# Autodesk Inventor assembly: Drivebase AM14U4 Square 28inx28in v411
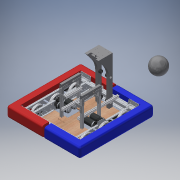
[picture p0: Inventor's stored thumbnail of the model, 180x180]
Saved by Autodesk Inventor 2018 (Build 220112000, 112)
## iProperties
Created: 2020-01-28
Part Number: Drivebase AM14U4 Square 28inx28in v411
Document SubType Name: Assembly
Designer: Weeb No1
Sending System: Autodesk Translation Framework v8.12.0.6
Preprocessor: ST-DEVELOPER v18
Title: /Users/GabG/Documents/GitHub/2020CAD/New Gabriel Shooter/Drivebase AM14U4 Square 28inx28in v41.step
## Documents named in this file (18)
- C:\Users\Weeb No1\Documents\GitHub\2020CAD\Gabriel Inventor Files (Shooter, Drivebase)\Drivebase Assembly\Main Assembly\Drivebase AM14U4 Square 28inx28in v411.iam
- C:\Users\Weeb No1\Documents\GitHub\2020CAD\Gabriel Inventor Files (Shooter, Drivebase)\Drivebase Assembly\Part Files\AM14U4 Square Half.iam
- C:\Users\Weeb No1\Documents\GitHub\2020CAD\Gabriel Inventor Files (Shooter, Drivebase)\Drivebase Assembly\Part Files\AM14U4 Square Half_1.iam
- C:\Users\Weeb No1\Documents\GitHub\2020CAD\Gabriel Inventor Files (Shooter, Drivebase)\Drivebase Assembly\Part Files\Placeholder Belly Pan.ipt
- C:\Users\Weeb No1\Documents\GitHub\2020CAD\Gabriel Inventor Files (Shooter, Drivebase)\Drivebase Assembly\Part Files\10-24 Washer.ipt
- C:\Users\Weeb No1\Documents\GitHub\2020CAD\Gabriel Inventor Files (Shooter, Drivebase)\Drivebase Assembly\Part Files\Bumper Assembly.iam
- C:\Users\Weeb No1\Documents\GitHub\2020CAD\Gabriel Inventor Files (Shooter, Drivebase)\Drivebase Assembly\Part Files\Bumper Assembly_1.iam
- C:\Users\Weeb No1\Documents\GitHub\2020CAD\Gabriel Inventor Files (Shooter, Drivebase)\Drivebase Assembly\Part Files\95335A503_METRIC QUICK-RELEASE PIN.ipt
- C:\Users\Weeb No1\Documents\GitHub\2020CAD\Gabriel Inventor Files (Shooter, Drivebase)\Drivebase Assembly\Part Files\8020 1010 x 19 v2.ipt
- C:\Users\Weeb No1\Documents\GitHub\2020CAD\Gabriel Inventor Files (Shooter, Drivebase)\Drivebase Assembly\Part Files\8020 1010 x 11 5 v2.ipt
- C:\Users\Weeb No1\Documents\GitHub\2020CAD\Gabriel Inventor Files (Shooter, Drivebase)\Drivebase Assembly\Part Files\1x2 9in 1_16_ Beam v7.ipt
- C:\Users\Weeb No1\Documents\GitHub\2020CAD\Gabriel Inventor Files (Shooter, Drivebase)\Drivebase Assembly\Part Files\L-Guesset v1.ipt
- C:\Users\Weeb No1\Documents\GitHub\2020CAD\Gabriel Inventor Files (Shooter, Drivebase)\Drivebase Assembly\Part Files\L-Bracket v1.ipt
- C:\Users\Weeb No1\Documents\GitHub\2020CAD\Gabriel Inventor Files (Shooter, Drivebase)\Drivebase Assembly\Part Files\Component52.ipt
- C:\Users\Weeb No1\Documents\GitHub\2020CAD\Gabriel Inventor Files (Shooter, Drivebase)\Drivebase Assembly\Part Files\8020 1010 x 8 7_8 v6.ipt
- C:\Users\Weeb No1\Documents\GitHub\2020CAD\Gabriel Inventor Files (Shooter, Drivebase)\Drivebase Assembly\Part Files\am-2986 FR8ZZ Hex Bearing v1.ipt
- C:\Users\Weeb No1\Documents\GitHub\2020CAD\Gabriel Inventor Files (Shooter, Drivebase)\Drivebase Assembly\Part Files\Clamping_Shaft_Collar_-_1_2_Hex_ID_217-2737 v1.ipt
- C:\Users\Weeb No1\Documents\GitHub\2020CAD\Gabriel Inventor Files (Shooter, Drivebase)\3D Printed Curve Assembly\Main Assembly\Solid Curve 3D Print v25.iam
## Components (54 placed, 17 different names)
1. AM14U4 Square Half:1 [sub-assembly] — Mate:1, Flush:2, Flush:1, Mate:2, Flush:4, Flush:3, Mate:62, Mate:63, Flush:42, Mate:64, Mate:65, Flush:43, Mate:69, Mate:70, Mate:71, Mate:75, Mate:76, Mate:77, Mate:82, Mate:83, Mate:84, Mate:85, Mate:91, Mate:92, Mate:96, Mate:97
2. AM14U4 Square Half_1:1 [sub-assembly] — Mate:66, Mate:67, Mate:68, Mate:72, Mate:73, Mate:74, Mate:78, Mate:79, Mate:80, Mate:81, Mate:93, Mate:94, Mate:95, Mate:98
3. Placeholder Belly Pan:1 — Mate:21, Mate:59, Mate:22, Mate:58, Mate:86, Mate:91, Mate:92, Mate:93, Mate:94, Mate:95, Mate:96, Mate:97, Mate:98, Mate:99, Mate:100, Mate:101, Mate:102, Mate:103, Mate:104, Mate:105, Mate:106
4. 10-24 Washer:1 — Mate:101
5. 10-24 Washer:2 — Mate:102
6. 10-24 Washer:3 — Mate:100
7. 10-24 Washer:4 — Mate:99
8. 10-24 Washer:5 — Mate:106
9. 10-24 Washer:6 — Mate:105
10. 10-24 Washer:7 — Mate:104
11. 10-24 Washer:8 — Mate:103
12. Bumper Assembly:1 [sub-assembly] — Mate:72, Mate:73, Mate:74, Mate:75, Mate:76, Mate:77
13. Bumper Assembly_1:1 [sub-assembly] — Mate:66, Mate:67, Mate:68, Mate:69, Mate:70, Mate:71
14. 95335A503_METRIC QUICK-RELEASE PIN:1 — Mate:82
15. 95335A503_METRIC QUICK-RELEASE PIN:2 — Mate:83
16. 95335A503_METRIC QUICK-RELEASE PIN:3 — Mate:85
17. 95335A503_METRIC QUICK-RELEASE PIN:4 — Mate:84
18. 95335A503_METRIC QUICK-RELEASE PIN:5 — Mate:78
19. 95335A503_METRIC QUICK-RELEASE PIN:6 — Mate:79
20. 95335A503_METRIC QUICK-RELEASE PIN:7 — Mate:80
21. 95335A503_METRIC QUICK-RELEASE PIN:8 — Mate:81
22. 8020 1010 x 19 v2:1 — Mate:1, Flush:2, Flush:1, Flush:17, Mate:20, Mate:19, Mate:87, Mate:110
23. 8020 1010 x 19 v2:2 — Mate:2, Flush:4, Flush:3, Mate:60, Flush:41, Mate:61, Mate:88, Mate:108
24. 8020 1010 x 11 5 v2:1 — Mate:21, Flush:17, Mate:20, Mate:18, Flush:16, Flush:15, Flush:18, Mate:25, Mate:109, Flush:45
25. 8020 1010 x 11 5 v2:2 — Mate:60, Flush:41, Mate:59, Flush:39, Flush:38, Mate:56, Mate:55, Flush:23, Mate:32, Mate:107, Flush:44
26. 8020 1010 x 11 5 v2:3 — Mate:22, Mate:19, Flush:14, Flush:13, Mate:17, Flush:21, Mate:29
27. 1x2 9in 1_16_ Beam v7:1 — Mate:18, Flush:16, Flush:15, Flush:14, Flush:13, Mate:17, Mate:8, Mate:7, Mate:6, Flush:8, Flush:7, Mate:14, Mate:13, Mate:12, Flush:12, Flush:11, Flush:32, Flush:31, Mate:5, Mate:4, Mate:3, Flush:6, Flush:5, Mate:11, Mate:10, Mate:9, Flush:10, Flush:9, Mate:16, Mate:15
28. 8020 1010 x 11 5 v2:4 — Mate:61, Mate:58, Flush:40, Flush:37, Mate:57, Flush:28, Mate:37
29. 1x2 9in 1_16_ Beam v7:2 — Flush:40, Flush:39, Flush:38, Flush:37, Mate:57, Mate:56, Mate:55, Flush:34, Flush:33, Mate:51, Mate:50, Mate:49, Flush:36, Flush:35, Mate:54, Mate:53, Mate:52, Mate:48, Mate:47, Mate:46, Flush:30, Flush:29, Mate:45, Mate:44, Mate:43, Mate:40, Mate:39
30. L-Guesset v1:1 — Flush:18, Mate:25, Flush:19, Mate:27, Mate:26, Mate:24, Mate:23
31. L-Bracket v1:1 — Flush:19, Mate:27, Mate:26, Flush:20, Mate:28
32. L-Guesset v1:2 — Flush:23, Mate:32, Flush:26, Mate:34, Flush:24, Mate:33
33. L-Bracket v1:2 — Flush:26, Mate:34, Flush:25, Mate:35
34. L-Guesset v1:3 — Mate:8, Mate:7, Mate:6, Flush:8, Flush:7
35. L-Guesset v1:4 — Mate:14, Mate:13, Mate:12, Flush:12, Flush:11
36. L-Guesset v1:5 — Flush:34, Flush:33, Mate:51, Mate:50, Mate:49
37. L-Guesset v1:6 — Flush:36, Flush:35, Mate:54, Mate:53, Mate:52
38. L-Guesset v1:7 — Flush:32, Flush:31, Mate:5, Mate:4, Mate:3, Flush:6, Flush:5
39. L-Guesset v1:8 — Mate:11, Mate:10, Mate:9, Flush:10, Flush:9
40. L-Guesset v1:9 — Mate:48, Mate:47, Mate:46
41. L-Guesset v1:10 — Flush:30, Flush:29, Mate:45, Mate:44, Mate:43
42. L-Bracket v1:3 — Mate:107, Mate:108, Flush:44
43. L-Bracket v1:4 — Mate:109, Mate:110, Flush:45
44. Component52:1
45. L-Guesset v1:11 — Flush:21, Mate:29, Flush:22, Mate:31, Mate:30
46. L-Guesset v1:12 — Flush:28, Mate:37, Flush:27, Mate:38, Mate:36
47. L-Bracket v1:7 — Mate:62, Mate:63, Flush:42, Mate:89
48. L-Bracket v1:8 — Mate:64, Mate:65, Flush:43, Mate:90
49. 8020 1010 x 8 7_8 v6:1 — Flush:27, Mate:38, Mate:36, Flush:25, Mate:35, Flush:24, Mate:33
50. 8020 1010 x 8 7_8 v6:2 — Flush:22, Mate:31, Mate:30, Flush:20, Mate:28, Mate:24, Mate:23
51. am-2986 FR8ZZ Hex Bearing v1:1 — Mate:40, Mate:39, Mate:42, Mate:41
52. Clamping_Shaft_Collar_-_1_2_Hex_ID_217-2737 v1:1 — Mate:42, Mate:41
53. am-2986 FR8ZZ Hex Bearing v1:2 — Mate:16, Mate:15
54. Solid Curve 3D Print v25:1 [sub-assembly] — Mate:86, Mate:87, Mate:88, Mate:89, Mate:90
## Relationships (155: Mate 110, Flush 45)
- Mate:1: AM14U4 Square Half:1 ↔ 8020 1010 x 19 v2:1
- Flush:2 (247.65 mm): AM14U4 Square Half:1 ↔ 8020 1010 x 19 v2:1
- Flush:1: AM14U4 Square Half:1 ↔ 8020 1010 x 19 v2:1
- Mate:2: AM14U4 Square Half:1 ↔ 8020 1010 x 19 v2:2
- Flush:4 (247.65 mm): AM14U4 Square Half:1 ↔ 8020 1010 x 19 v2:2
- Flush:3: AM14U4 Square Half:1 ↔ 8020 1010 x 19 v2:2
- Mate:21: Placeholder Belly Pan:1 ↔ 8020 1010 x 11 5 v2:1
- Flush:17 (9.525 mm): 8020 1010 x 19 v2:1 ↔ 8020 1010 x 11 5 v2:1
- Mate:20: 8020 1010 x 19 v2:1 ↔ 8020 1010 x 11 5 v2:1
- Mate:60: 8020 1010 x 19 v2:2 ↔ 8020 1010 x 11 5 v2:2
- Flush:41 (9.525 mm): 8020 1010 x 19 v2:2 ↔ 8020 1010 x 11 5 v2:2
- Mate:59: Placeholder Belly Pan:1 ↔ 8020 1010 x 11 5 v2:2
- Mate:22: Placeholder Belly Pan:1 ↔ 8020 1010 x 11 5 v2:3
- Mate:19: 8020 1010 x 19 v2:1 ↔ 8020 1010 x 11 5 v2:3
- Mate:18: 8020 1010 x 11 5 v2:1 ↔ 1x2 9in 1_16_ Beam v7:1
- Flush:16: 8020 1010 x 11 5 v2:1 ↔ 1x2 9in 1_16_ Beam v7:1
- Flush:15: 8020 1010 x 11 5 v2:1 ↔ 1x2 9in 1_16_ Beam v7:1
- Flush:14: 8020 1010 x 11 5 v2:3 ↔ 1x2 9in 1_16_ Beam v7:1
- Flush:13: 8020 1010 x 11 5 v2:3 ↔ 1x2 9in 1_16_ Beam v7:1
- Mate:17: 8020 1010 x 11 5 v2:3 ↔ 1x2 9in 1_16_ Beam v7:1
- Mate:61: 8020 1010 x 19 v2:2 ↔ 8020 1010 x 11 5 v2:4
- Mate:58: Placeholder Belly Pan:1 ↔ 8020 1010 x 11 5 v2:4
- Flush:40: 8020 1010 x 11 5 v2:4 ↔ 1x2 9in 1_16_ Beam v7:2
- Flush:39: 8020 1010 x 11 5 v2:2 ↔ 1x2 9in 1_16_ Beam v7:2
- Flush:38: 8020 1010 x 11 5 v2:2 ↔ 1x2 9in 1_16_ Beam v7:2
- Flush:37: 8020 1010 x 11 5 v2:4 ↔ 1x2 9in 1_16_ Beam v7:2
- Mate:57: 8020 1010 x 11 5 v2:4 ↔ 1x2 9in 1_16_ Beam v7:2
- Mate:56: 8020 1010 x 11 5 v2:2 ↔ 1x2 9in 1_16_ Beam v7:2
- Mate:55: 8020 1010 x 11 5 v2:2 ↔ 1x2 9in 1_16_ Beam v7:2
- Flush:18: 8020 1010 x 11 5 v2:1 ↔ L-Guesset v1:1
- Mate:25: 8020 1010 x 11 5 v2:1 ↔ L-Guesset v1:1
- Flush:19: L-Guesset v1:1 ↔ L-Bracket v1:1
- Mate:27: L-Guesset v1:1 ↔ L-Bracket v1:1
- Mate:26: L-Guesset v1:1 ↔ L-Bracket v1:1
- Flush:23: 8020 1010 x 11 5 v2:2 ↔ L-Guesset v1:2
- Mate:32: 8020 1010 x 11 5 v2:2 ↔ L-Guesset v1:2
- Flush:26: L-Guesset v1:2 ↔ L-Bracket v1:2
- Mate:34: L-Guesset v1:2 ↔ L-Bracket v1:2
- Mate:8: 1x2 9in 1_16_ Beam v7:1 ↔ L-Guesset v1:3
- Mate:7: 1x2 9in 1_16_ Beam v7:1 ↔ L-Guesset v1:3
- Mate:6: 1x2 9in 1_16_ Beam v7:1 ↔ L-Guesset v1:3
- Flush:8: 1x2 9in 1_16_ Beam v7:1 ↔ L-Guesset v1:3
- Flush:7: 1x2 9in 1_16_ Beam v7:1 ↔ L-Guesset v1:3
- Mate:14: 1x2 9in 1_16_ Beam v7:1 ↔ L-Guesset v1:4
- Mate:13: 1x2 9in 1_16_ Beam v7:1 ↔ L-Guesset v1:4
- Mate:12: 1x2 9in 1_16_ Beam v7:1 ↔ L-Guesset v1:4
- Flush:12: 1x2 9in 1_16_ Beam v7:1 ↔ L-Guesset v1:4
- Flush:11: 1x2 9in 1_16_ Beam v7:1 ↔ L-Guesset v1:4
- Flush:34: 1x2 9in 1_16_ Beam v7:2 ↔ L-Guesset v1:5
- Flush:33: 1x2 9in 1_16_ Beam v7:2 ↔ L-Guesset v1:5
- Mate:51: 1x2 9in 1_16_ Beam v7:2 ↔ L-Guesset v1:5
- Mate:50: 1x2 9in 1_16_ Beam v7:2 ↔ L-Guesset v1:5
- Mate:49: 1x2 9in 1_16_ Beam v7:2 ↔ L-Guesset v1:5
- Flush:36: 1x2 9in 1_16_ Beam v7:2 ↔ L-Guesset v1:6
- Flush:35: 1x2 9in 1_16_ Beam v7:2 ↔ L-Guesset v1:6
- Mate:54: 1x2 9in 1_16_ Beam v7:2 ↔ L-Guesset v1:6
- Mate:53: 1x2 9in 1_16_ Beam v7:2 ↔ L-Guesset v1:6
- Mate:52: 1x2 9in 1_16_ Beam v7:2 ↔ L-Guesset v1:6
- Flush:32: 1x2 9in 1_16_ Beam v7:1 ↔ L-Guesset v1:7
- Flush:31: 1x2 9in 1_16_ Beam v7:1 ↔ L-Guesset v1:7
- Mate:5: 1x2 9in 1_16_ Beam v7:1 ↔ L-Guesset v1:7
- Mate:4: 1x2 9in 1_16_ Beam v7:1 ↔ L-Guesset v1:7
- Mate:3: 1x2 9in 1_16_ Beam v7:1 ↔ L-Guesset v1:7
- Flush:6: 1x2 9in 1_16_ Beam v7:1 ↔ L-Guesset v1:7
- Flush:5: 1x2 9in 1_16_ Beam v7:1 ↔ L-Guesset v1:7
- Mate:11: 1x2 9in 1_16_ Beam v7:1 ↔ L-Guesset v1:8
- Mate:10: 1x2 9in 1_16_ Beam v7:1 ↔ L-Guesset v1:8
- Mate:9: 1x2 9in 1_16_ Beam v7:1 ↔ L-Guesset v1:8
- Flush:10: 1x2 9in 1_16_ Beam v7:1 ↔ L-Guesset v1:8
- Flush:9: 1x2 9in 1_16_ Beam v7:1 ↔ L-Guesset v1:8
- Mate:48: 1x2 9in 1_16_ Beam v7:2 ↔ L-Guesset v1:9
- Mate:47: 1x2 9in 1_16_ Beam v7:2 ↔ L-Guesset v1:9
- Mate:46: 1x2 9in 1_16_ Beam v7:2 ↔ L-Guesset v1:9
- Flush:30: 1x2 9in 1_16_ Beam v7:2 ↔ L-Guesset v1:10
- Flush:29: 1x2 9in 1_16_ Beam v7:2 ↔ L-Guesset v1:10
- Mate:45: 1x2 9in 1_16_ Beam v7:2 ↔ L-Guesset v1:10
- Mate:44: 1x2 9in 1_16_ Beam v7:2 ↔ L-Guesset v1:10
- Mate:43: 1x2 9in 1_16_ Beam v7:2 ↔ L-Guesset v1:10
- Flush:21: 8020 1010 x 11 5 v2:3 ↔ L-Guesset v1:11
- Mate:29: 8020 1010 x 11 5 v2:3 ↔ L-Guesset v1:11
- Flush:28: 8020 1010 x 11 5 v2:4 ↔ L-Guesset v1:12
- Mate:37: 8020 1010 x 11 5 v2:4 ↔ L-Guesset v1:12
- Flush:27: L-Guesset v1:12 ↔ 8020 1010 x 8 7_8 v6:1
- Mate:38: L-Guesset v1:12 ↔ 8020 1010 x 8 7_8 v6:1
- Mate:36: L-Guesset v1:12 ↔ 8020 1010 x 8 7_8 v6:1
- Flush:25: L-Bracket v1:2 ↔ 8020 1010 x 8 7_8 v6:1
- Mate:35: L-Bracket v1:2 ↔ 8020 1010 x 8 7_8 v6:1
- Flush:24: L-Guesset v1:2 ↔ 8020 1010 x 8 7_8 v6:1
- Mate:33: L-Guesset v1:2 ↔ 8020 1010 x 8 7_8 v6:1
- Flush:22: L-Guesset v1:11 ↔ 8020 1010 x 8 7_8 v6:2
- Mate:31: L-Guesset v1:11 ↔ 8020 1010 x 8 7_8 v6:2
- Mate:30: L-Guesset v1:11 ↔ 8020 1010 x 8 7_8 v6:2
- Flush:20: L-Bracket v1:1 ↔ 8020 1010 x 8 7_8 v6:2
- Mate:28: L-Bracket v1:1 ↔ 8020 1010 x 8 7_8 v6:2
- Mate:24: L-Guesset v1:1 ↔ 8020 1010 x 8 7_8 v6:2
- Mate:23: L-Guesset v1:1 ↔ 8020 1010 x 8 7_8 v6:2
- Mate:40: 1x2 9in 1_16_ Beam v7:2 ↔ am-2986 FR8ZZ Hex Bearing v1:1
- Mate:39: 1x2 9in 1_16_ Beam v7:2 ↔ am-2986 FR8ZZ Hex Bearing v1:1
- Mate:42: am-2986 FR8ZZ Hex Bearing v1:1 ↔ Clamping_Shaft_Collar_-_1_2_Hex_ID_217-2737 v1:1
- Mate:41: am-2986 FR8ZZ Hex Bearing v1:1 ↔ Clamping_Shaft_Collar_-_1_2_Hex_ID_217-2737 v1:1
- Mate:16: 1x2 9in 1_16_ Beam v7:1 ↔ am-2986 FR8ZZ Hex Bearing v1:2
- Mate:15: 1x2 9in 1_16_ Beam v7:1 ↔ am-2986 FR8ZZ Hex Bearing v1:2
- Mate:62: AM14U4 Square Half:1 ↔ L-Bracket v1:7
- Mate:63: AM14U4 Square Half:1 ↔ L-Bracket v1:7
- Flush:42 (-0.762 mm): AM14U4 Square Half:1 ↔ L-Bracket v1:7
- Mate:64: AM14U4 Square Half:1 ↔ L-Bracket v1:8
- Mate:65: AM14U4 Square Half:1 ↔ L-Bracket v1:8
- Flush:43 (-0.762 mm): AM14U4 Square Half:1 ↔ L-Bracket v1:8
- Mate:66: AM14U4 Square Half_1:1 ↔ Bumper Assembly_1:1
- Mate:67: AM14U4 Square Half_1:1 ↔ Bumper Assembly_1:1
- Mate:68: AM14U4 Square Half_1:1 ↔ Bumper Assembly_1:1
- Mate:69: AM14U4 Square Half:1 ↔ Bumper Assembly_1:1
- Mate:70: AM14U4 Square Half:1 ↔ Bumper Assembly_1:1
- Mate:71: AM14U4 Square Half:1 ↔ Bumper Assembly_1:1
- Mate:72: AM14U4 Square Half_1:1 ↔ Bumper Assembly:1
- Mate:73: AM14U4 Square Half_1:1 ↔ Bumper Assembly:1
- Mate:74: AM14U4 Square Half_1:1 ↔ Bumper Assembly:1
- Mate:75: AM14U4 Square Half:1 ↔ Bumper Assembly:1
- Mate:76: AM14U4 Square Half:1 ↔ Bumper Assembly:1
- Mate:77: AM14U4 Square Half:1 ↔ Bumper Assembly:1
- Mate:78: AM14U4 Square Half_1:1 ↔ 95335A503_METRIC QUICK-RELEASE PIN:5
- Mate:79: AM14U4 Square Half_1:1 ↔ 95335A503_METRIC QUICK-RELEASE PIN:6
- Mate:80: AM14U4 Square Half_1:1 ↔ 95335A503_METRIC QUICK-RELEASE PIN:7
- Mate:81: AM14U4 Square Half_1:1 ↔ 95335A503_METRIC QUICK-RELEASE PIN:8
- Mate:82: AM14U4 Square Half:1 ↔ 95335A503_METRIC QUICK-RELEASE PIN:1
- Mate:83: AM14U4 Square Half:1 ↔ 95335A503_METRIC QUICK-RELEASE PIN:2
- Mate:84: AM14U4 Square Half:1 ↔ 95335A503_METRIC QUICK-RELEASE PIN:4
- Mate:85: AM14U4 Square Half:1 ↔ 95335A503_METRIC QUICK-RELEASE PIN:3
- Mate:86: Placeholder Belly Pan:1 ↔ Solid Curve 3D Print v25:1
- Mate:87: 8020 1010 x 19 v2:1 ↔ Solid Curve 3D Print v25:1
- Mate:88: 8020 1010 x 19 v2:2 ↔ Solid Curve 3D Print v25:1
- Mate:89: L-Bracket v1:7 ↔ Solid Curve 3D Print v25:1
- Mate:90: L-Bracket v1:8 ↔ Solid Curve 3D Print v25:1
- Mate:91: AM14U4 Square Half:1 ↔ Placeholder Belly Pan:1
- Mate:92: AM14U4 Square Half:1 ↔ Placeholder Belly Pan:1
- Mate:93: AM14U4 Square Half_1:1 ↔ Placeholder Belly Pan:1
- Mate:94: AM14U4 Square Half_1:1 ↔ Placeholder Belly Pan:1
- Mate:95: AM14U4 Square Half_1:1 ↔ Placeholder Belly Pan:1
- Mate:96: AM14U4 Square Half:1 ↔ Placeholder Belly Pan:1
- Mate:97: AM14U4 Square Half:1 ↔ Placeholder Belly Pan:1
- Mate:98: AM14U4 Square Half_1:1 ↔ Placeholder Belly Pan:1
- Mate:99: Placeholder Belly Pan:1 ↔ 10-24 Washer:4
- Mate:100: Placeholder Belly Pan:1 ↔ 10-24 Washer:3
- Mate:101: Placeholder Belly Pan:1 ↔ 10-24 Washer:1
- Mate:102: Placeholder Belly Pan:1 ↔ 10-24 Washer:2
- Mate:103: Placeholder Belly Pan:1 ↔ 10-24 Washer:8
- Mate:104: Placeholder Belly Pan:1 ↔ 10-24 Washer:7
- Mate:105: Placeholder Belly Pan:1 ↔ 10-24 Washer:6
- Mate:106: Placeholder Belly Pan:1 ↔ 10-24 Washer:5
- Mate:107: 8020 1010 x 11 5 v2:2 ↔ L-Bracket v1:3
- Mate:108: 8020 1010 x 19 v2:2 ↔ L-Bracket v1:3
- Flush:44: 8020 1010 x 11 5 v2:2 ↔ L-Bracket v1:3
- Mate:109: 8020 1010 x 11 5 v2:1 ↔ L-Bracket v1:4
- Mate:110: 8020 1010 x 19 v2:1 ↔ L-Bracket v1:4
- Flush:45: 8020 1010 x 11 5 v2:1 ↔ L-Bracket v1:4
